# Autodesk Inventor assembly: OktagonElektronik_Stage3
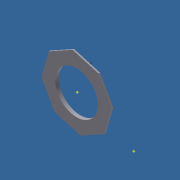
[picture p0: Inventor's stored thumbnail of the model, 180x180]
Saved by Autodesk Inventor 2018.2 (Build 222227000, 227)
## iProperties
Company: Fraunhofer ILT
Created: 2018-10-31
Part Number: OktagonElektronik_Stage3
Material: geeigneten Werkstoff auswählen !
Document SubType Name: Assembly
Designer: N.Grubert
Title: =Description
Author: N.Grubert
## Documents named in this file (3)
- C:\Users\GRUBERT\Documents\COSIMA-Laserstar\CAD\Oktokommander\OktagonElektronik_Stage3.iam
- C:\Users\GRUBERT\Documents\COSIMA-Laserstar\CAD\Oktokommander\Stage3.ipt
- C:\Users\GRUBERT\Documents\COSIMA-Laserstar\CAD\Oktokommander\Photodiodendummie.ipt
## Components (5 placed, 2 different names)
1. Stage3:1 — Passend:1, Passend:2, Passend:3, Passend:4, Passend:5, Passend:6, Passend:7, Passend:8
2. Photodiodendummie:1 — Passend:4, Passend:7
3. Photodiodendummie:2 — Passend:2, Passend:5
4. Photodiodendummie:3 — Passend:1, Passend:6
5. Photodiodendummie:4 — Passend:3, Passend:8
## Relationships (8: Mate 8)
- Passend:1 [Mate]: Stage3:1 ↔ Photodiodendummie:3
- Passend:2 [Mate]: Stage3:1 ↔ Photodiodendummie:2
- Passend:3 [Mate]: Stage3:1 ↔ Photodiodendummie:4
- Passend:4 [Mate]: Stage3:1 ↔ Photodiodendummie:1
- Passend:5 [Mate]: Stage3:1 ↔ Photodiodendummie:2
- Passend:6 [Mate]: Stage3:1 ↔ Photodiodendummie:3
- Passend:7 [Mate]: Stage3:1 ↔ Photodiodendummie:1
- Passend:8 [Mate]: Stage3:1 ↔ Photodiodendummie:4
